# Autodesk Inventor assembly: CAJA_ENGRANAJES_COMPLETA
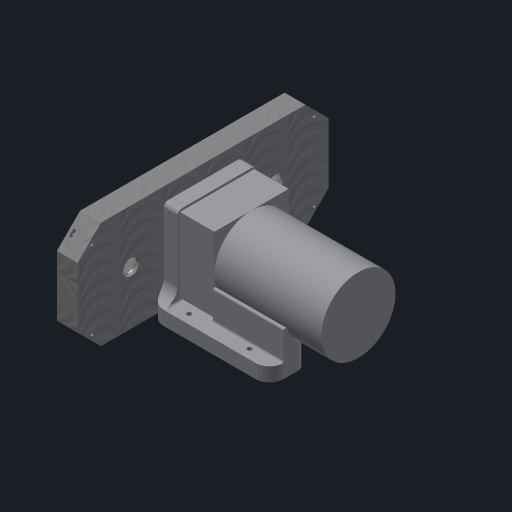
[picture p0: Inventor's stored thumbnail of the model, 512x512]
Saved by Autodesk Inventor 2024.3 (Build 283343000, 343)
## iProperties
Created: 2024-06-29
Part Number: CAJA_ENGRANAJES_COMPLETA
Material: Generic
Document SubType Name: Assembly
Designer: Niler
Author: Niler
## Documents named in this file (14)
- C:\Users\Niler\OneDrive\Escritorio\RECICLADOR\RECICLADOR_MODELO_3D\CAJA_ENGRANAJES\VERSION_3\CAJA_ENGRANAJES_COMPLETA_V3.iam
- C:\Users\Niler\OneDrive\Escritorio\RECICLADOR\RECICLADOR_MODELO_3D\CAJA_ENGRANAJES\CAJA_ENGRANAJES_COMPLETA\Design Accelerator\Bearing1.iam
- C:\Users\Niler\OneDrive\Escritorio\RECICLADOR\RECICLADOR_MODELO_3D\LIBRERIA\en-US\ANSI B18.2.4.2M\ANSI B18.2.4.2M - M8x1.25 - 13.ipt
- C:\Users\Niler\OneDrive\Escritorio\RECICLADOR\RECICLADOR_MODELO_3D\CAJA_ENGRANAJES\VERSION_3\ENGRANAJES_V3\Design Accelerator\Spur Gear11.ipt
- C:\Users\Niler\OneDrive\Escritorio\RECICLADOR\RECICLADOR_MODELO_3D\CAJA_ENGRANAJES\VERSION_3\ENGRANAJES_V3\Design Accelerator\Spur Gear21.ipt
- C:\Users\Niler\OneDrive\Escritorio\RECICLADOR\RECICLADOR_MODELO_3D\LIBRERIA\en-US\AS 1237 (3.1)\AS 1237 - 8 mm(1)Aluminium-6061.ipt
- C:\Users\Niler\OneDrive\Escritorio\RECICLADOR\RECICLADOR_MODELO_3D\CAJA_ENGRANAJES\VERSION_3\CAJA_V3.ipt
- C:\Users\Niler\OneDrive\Escritorio\RECICLADOR\RECICLADOR_MODELO_3D\CAJA_ENGRANAJES\VERSION_3\CAJA_P2_V3.ipt
- C:\Users\Niler\OneDrive\Escritorio\RECICLADOR\RECICLADOR_MODELO_3D\LIBRERIA\en-US\DIN 976-1 A\DIN 976-1 - M8 x 50 - A.ipt
- C:\Users\Niler\OneDrive\Escritorio\RECICLADOR\RECICLADOR_MODELO_3D\MECANISMO DE COMPACTADO\SOPORTE DEL MOTOR.ipt
- C:\Users\Niler\OneDrive\Escritorio\RECICLADOR\RECICLADOR_MODELO_3D\MECANISMO DE COMPACTADO\MOTOR DC.ipt
- C:\Users\Niler\OneDrive\Escritorio\RECICLADOR\RECICLADOR_MODELO_3D\CAJA_ENGRANAJES\VERSION_3\RODAMIENTO_19X10X5.ipt
- C:\Users\Niler\OneDrive\Escritorio\RECICLADOR\RECICLADOR_MODELO_3D\LIBRERIA\en-US\AS 1237 (3.1)\AS 1237 - 10 mm(1)Aluminium-6061.ipt
- C:\Users\Niler\OneDrive\Escritorio\RECICLADOR\RECICLADOR_MODELO_3D\CAJA_ENGRANAJES\VERSION_3\PIEZA_AYUDA.ipt
## Components (22 placed, 13 different names)
1. CAJA_V3:1 — Mate:39, Mate:40, Mate:42, Mate:43, Flush:3, Flush:4, Mate:48, Mate:51, Mate:52, Mate:53, Mate:56
2. ANSI B18.2.4.2M M8x1.25:1 — Mate:15, Mate:18, Mate:21
3. Spur Gear1:1 — Mate:59, Mate:63
4. Spur Gear2:1 — Mate:15, Mate:22, Mate:23, Flush:1, Mate:36
5. AS 1237 (3.1) 8 mm - Aluminum 6061:1 — Mate:18, Mate:20, Mate:22, Mate:29
6. DIN 976-1 A M8 x 50:1 — Mate:20, Mate:21, Mate:23, Flush:1, Mate:33, Mate:41
7. Bearing:3 [sub-assembly] — Mate:29, Mate:39, Mate:40, Mate:41
8. Bearing:4 [sub-assembly] — Mate:37, Mate:38, Mate:42, Mate:43
9. Spur Gear2:2 — Mate:35
10. AS 1237 (3.1) 8 mm - Aluminum 6061:2 — Mate:38
11. DIN 976-1 A M8 x 50:2 — Mate:34, Mate:37
12. AS 1237 (3.1) 8 mm - Aluminum 6061:3 — Mate:33, Mate:36
13. AS 1237 (3.1) 8 mm - Aluminum 6061:4 — Mate:34, Mate:35
14. CAJA_P2_V3:1 — Flush:3, Flush:4, Mate:44, Mate:45, Mate:46, Mate:47, Mate:48, Mate:60, Mate:61
15. Bearing:5 [sub-assembly] — Mate:44, Mate:47
16. Bearing:6 [sub-assembly] — Mate:45, Mate:46
17. SOPORTE DEL MOTOR:1 — Mate:51, Mate:52, Mate:53, Angle:1
18. MOTOR DC:1 — Angle:1, Mate:55, Mate:57
19. RODAMIENTO_19X10X5:1 — Mate:55, Mate:56, Mate:58
20. AS 1237 (3.1) 10 mm - Aluminum 6061:1 — Mate:57, Mate:58, Mate:59
21. RODAMIENTO_19X10X5:2 — Mate:60, Mate:61, Mate:62
22. PIEZA_AYUDA:1 — Mate:62, Mate:63
## Relationships (45: Mate 40, Flush 4, Angle 1)
- Mate:15: ANSI B18.2.4.2M M8x1.25:1 ↔ Spur Gear2:1
- Mate:18: ANSI B18.2.4.2M M8x1.25:1 ↔ AS 1237 (3.1) 8 mm - Aluminum 6061:1
- Mate:20: AS 1237 (3.1) 8 mm - Aluminum 6061:1 ↔ DIN 976-1 A M8 x 50:1
- Mate:21: ANSI B18.2.4.2M M8x1.25:1 ↔ DIN 976-1 A M8 x 50:1
- Mate:22: Spur Gear2:1 ↔ AS 1237 (3.1) 8 mm - Aluminum 6061:1
- Mate:23: Spur Gear2:1 ↔ DIN 976-1 A M8 x 50:1
- Flush:1 (-8 mm): Spur Gear2:1 ↔ DIN 976-1 A M8 x 50:1
- Mate:29: AS 1237 (3.1) 8 mm - Aluminum 6061:1 ↔ Bearing:3
- [Mate]: AS 1237 (3.1) 8 mm - Aluminum 6061:2 ↔ DIN 976-1 A M8 x 50:2
- [Mate]: Spur Gear2:2 ↔ AS 1237 (3.1) 8 mm - Aluminum 6061:2
- [Mate]: Spur Gear2:2 ↔ DIN 976-1 A M8 x 50:2
- [Flush] (-8 mm): Spur Gear2:2 ↔ DIN 976-1 A M8 x 50:2
- Mate:33: DIN 976-1 A M8 x 50:1 ↔ AS 1237 (3.1) 8 mm - Aluminum 6061:3
- Mate:34: DIN 976-1 A M8 x 50:2 ↔ AS 1237 (3.1) 8 mm - Aluminum 6061:4
- Mate:35: Spur Gear2:2 ↔ AS 1237 (3.1) 8 mm - Aluminum 6061:4
- Mate:36: Spur Gear2:1 ↔ AS 1237 (3.1) 8 mm - Aluminum 6061:3
- Mate:37: Bearing:4 ↔ DIN 976-1 A M8 x 50:2
- Mate:38: Bearing:4 ↔ AS 1237 (3.1) 8 mm - Aluminum 6061:2
- Mate:39: CAJA_V3:1 ↔ Bearing:3
- Mate:40: CAJA_V3:1 ↔ Bearing:3
- Mate:41: DIN 976-1 A M8 x 50:1 ↔ Bearing:3
- Mate:42: CAJA_V3:1 ↔ Bearing:4
- Mate:43: CAJA_V3:1 ↔ Bearing:4
- Flush:3: CAJA_V3:1 ↔ CAJA_P2_V3:1
- Flush:4: CAJA_V3:1 ↔ CAJA_P2_V3:1
- Mate:44: CAJA_P2_V3:1 ↔ Bearing:5
- Mate:45: CAJA_P2_V3:1 ↔ Bearing:6
- Mate:46: CAJA_P2_V3:1 ↔ Bearing:6
- Mate:47: CAJA_P2_V3:1 ↔ Bearing:5
- Mate:48: CAJA_V3:1 ↔ CAJA_P2_V3:1
- [Mate]: SOPORTE DEL MOTOR:1 ↔ MOTOR DC:1
- [Mate]: SOPORTE DEL MOTOR:1 ↔ MOTOR DC:1
- Mate:51: CAJA_V3:1 ↔ SOPORTE DEL MOTOR:1
- Mate:52: CAJA_V3:1 ↔ SOPORTE DEL MOTOR:1
- Mate:53: CAJA_V3:1 ↔ SOPORTE DEL MOTOR:1
- Angle:1 (0 deg): SOPORTE DEL MOTOR:1 ↔ MOTOR DC:1
- Mate:55: MOTOR DC:1 ↔ RODAMIENTO_19X10X5:1
- Mate:56: CAJA_V3:1 ↔ RODAMIENTO_19X10X5:1
- Mate:57: MOTOR DC:1 ↔ AS 1237 (3.1) 10 mm - Aluminum 6061:1
- Mate:58: RODAMIENTO_19X10X5:1 ↔ AS 1237 (3.1) 10 mm - Aluminum 6061:1
- Mate:59: Spur Gear1:1 ↔ AS 1237 (3.1) 10 mm - Aluminum 6061:1
- Mate:60: CAJA_P2_V3:1 ↔ RODAMIENTO_19X10X5:2
- Mate:61: CAJA_P2_V3:1 ↔ RODAMIENTO_19X10X5:2
- Mate:62: RODAMIENTO_19X10X5:2 ↔ PIEZA_AYUDA:1
- Mate:63: Spur Gear1:1 ↔ PIEZA_AYUDA:1
## Named parameters: d53_d51 = -8 mm, d54_d44 = 0 mm, d55_d45 = 0 mm, d56_d42 = 0 mm
